# Autodesk Inventor assembly: Insert2
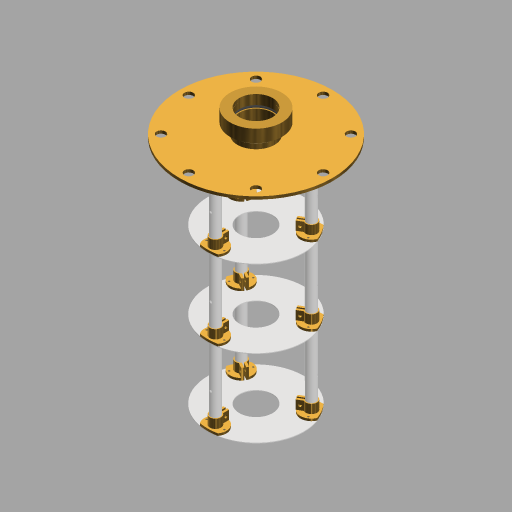
[picture p0: Inventor's stored thumbnail of the model, 512x512]
Saved by Autodesk Inventor 2024 (Build 280153020, 153B)
## iProperties
Created: 2023-10-26
Part Number: Insert2
Document SubType Name: Assembly
Designer: schanen
Mass: 2090.43 g
Surface Area: 3626.79 cm^2
Volume: 311.019 cm^3
Density: 6.72124 g/cm^3
Author: schanen
## Documents named in this file (5)
- C:\Users\schanen\Documents\Inventor\LargeTransportDewarInsert2023\Insert2.iam
- C:\Users\schanen\Documents\Inventor\LargeTransportDewarInsert2023\tube.ipt
- C:\Users\schanen\Documents\Inventor\LargeTransportDewarInsert2023\BaffleAssembly.iam
- C:\Users\schanen\Documents\Inventor\LargeTransportDewarInsert2023\tubeFitting.ipt
- C:\Users\schanen\Documents\Inventor\LargeTransportDewarInsert2023\Flange.iam
## Components (10 placed, 4 different names)
1. Flange:1 [sub-assembly] — Mate:11, Flush:1, Mate:14, Mate:15, Mate:16, Mate:17
2. tube:1 — Mate:6, Mate:7, Mate:10, Mate:16, Angle:1
3. tubeFitting:1 — Mate:6, Mate:7, Mate:14
4. tube:2
5. tubeFitting:2
6. tube:3
7. tubeFitting:3
8. BaffleAssembly:1 [sub-assembly] — Mate:10, Mate:12, Mate:15
9. BaffleAssembly:2 [sub-assembly]
10. BaffleAssembly:3 [sub-assembly]
## Component patterns: (3 elements, first: tube:1 + tubeFitting:1), (3 elements, first: BaffleAssembly:1)
## Relationships (11: Mate 9, Flush 1, Angle 1)
- Mate:6: tube:1 ↔ tubeFitting:1
- Mate:7: tube:1 ↔ tubeFitting:1
- Mate:10: tube:1 ↔ BaffleAssembly:1
- Mate:11: Flange:1
- Mate:12: BaffleAssembly:1
- Flush:1: Flange:1
- Mate:14: Flange:1 ↔ tubeFitting:1
- Mate:15 (100 mm): Flange:1 ↔ BaffleAssembly:1
- Mate:16: Flange:1 ↔ tube:1
- Mate:17: Flange:1
- Angle:1 (0 deg): tube:1
